# Autodesk Inventor assembly: Aki GS GTZ5S
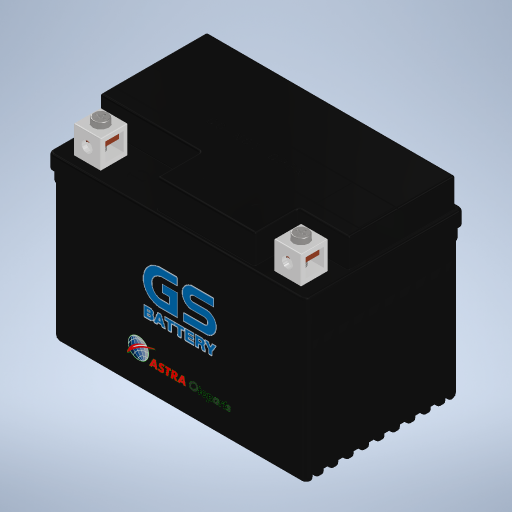
[picture p0: Inventor's stored thumbnail of the model, 512x512]
Saved by Autodesk Inventor 2023 (Build 270158000, 158)
## iProperties
Created: 2023-04-01
Part Number: Aki GS GTZ5S
Document SubType Name: Assembly
Designer: user
Author: user
## Documents named in this file (6)
- F:\Pindahan\Aki GS SEALED MF GTZ5S ASTRA Otoparts\Assembly Inventor\Aki GS GTZ5S.iam
- F:\Pindahan\Aki GS SEALED MF GTZ5S ASTRA Otoparts\Part Inventor\Badan Aki.ipt
- F:\Pindahan\Aki GS SEALED MF GTZ5S ASTRA Otoparts\Part Inventor\Tutup Aki.ipt
- F:\Pindahan\Aki GS SEALED MF GTZ5S ASTRA Otoparts\Part Inventor\Kutup Aki.ipt
- F:\Pindahan\Aki GS SEALED MF GTZ5S ASTRA Otoparts\Part Inventor\Ganjal Baut Kutup.ipt
- C:\Users\user\Documents\Inventor\Content Center Files\R2021\en-US\GB_T 822-2000 H\Screw GB_T 822 M4 x 10.ipt
## Components (8 placed, 5 different names)
1. Badan Aki:1 — Mate:1, Mate:2, Mate:3
2. Tutup Aki:1 — Mate:1, Mate:2, Mate:3, Insert:1, Insert:2, Mate:4, Mate:5
3. Kutup Aki:1 — Insert:2, Mate:5, Mate:7, Insert:4, Insert:5
4. Kutup Aki:2 — Insert:1, Mate:4, Mate:6, Insert:3, Insert:6
5. Ganjal Baut Kutup:1 — Mate:7, Insert:4
6. Ganjal Baut Kutup:2 — Mate:6, Insert:3
7. Screw GB/T 822-2000 Type H M4 x 10:1 — Insert:5
8. Screw GB/T 822-2000 Type H M4 x 10:2 — Insert:6
## Relationships (13: Mate 7, Insert 6)
- Mate:1: Badan Aki:1 ↔ Tutup Aki:1
- Mate:2: Badan Aki:1 ↔ Tutup Aki:1
- Mate:3: Badan Aki:1 ↔ Tutup Aki:1
- Insert:1: Tutup Aki:1 ↔ Kutup Aki:2
- Insert:2: Tutup Aki:1 ↔ Kutup Aki:1
- Mate:4: Tutup Aki:1 ↔ Kutup Aki:2
- Mate:5: Tutup Aki:1 ↔ Kutup Aki:1
- Mate:6: Kutup Aki:2 ↔ Ganjal Baut Kutup:2
- Mate:7: Kutup Aki:1 ↔ Ganjal Baut Kutup:1
- Insert:3: Kutup Aki:2 ↔ Ganjal Baut Kutup:2
- Insert:4: Kutup Aki:1 ↔ Ganjal Baut Kutup:1
- Insert:5: Kutup Aki:1 ↔ Screw GB/T 822-2000 Type H M4 x 10:1
- Insert:6: Kutup Aki:2 ↔ Screw GB/T 822-2000 Type H M4 x 10:2
